# Autodesk Inventor assembly: Complete back top housing
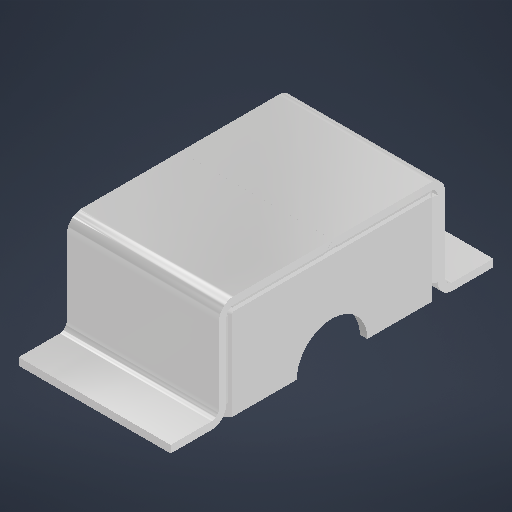
[picture p0: Inventor's stored thumbnail of the model, 512x512]
Saved by Autodesk Inventor 2026.3 (Build 303398000, 398)
## iProperties
Created: 2026-08-05
Part Number: Complete back top housing
Document SubType Name: Weldment
Designer: matot
Weld Material: Welded Aluminum-6061
Author: matot
## Documents named in this file (3)
- C:\Users\matot\OneDrive - Stellenbosch University\2026\MechatronicsProject478\Building the joint\Joint Assembly\Complete back top housing.iam
- C:\Users\matot\OneDrive - Stellenbosch University\2026\MechatronicsProject478\Building the joint\Joint Assembly\top front joint housing back.ipt
- C:\Users\matot\OneDrive - Stellenbosch University\2026\MechatronicsProject478\Building the joint\Joint Assembly\Bottom joint housing cover top back_ final.ipt
## Components (3 placed, 2 different names)
1. top front joint housing back:2 — Flush:1, Mate:1, Flush:2, Flush:3
2. top front joint housing back:3 — Flush:1, Mate:1, Flush:2, Flush:3, Mate:2, Mate:3, Flush:4
3. Bottom joint housing cover top back_ final:1 — Mate:2, Mate:3, Flush:4
## Relationships (7: Flush 4, Mate 3)
- Flush:1: top front joint housing back:2 ↔ top front joint housing back:3
- Mate:1: top front joint housing back:2 ↔ top front joint housing back:3
- Flush:2: top front joint housing back:2 ↔ top front joint housing back:3
- Flush:3: top front joint housing back:2 ↔ top front joint housing back:3
- Mate:2: top front joint housing back:3 ↔ Bottom joint housing cover top back_ final:1
- Mate:3: top front joint housing back:3 ↔ Bottom joint housing cover top back_ final:1
- Flush:4: top front joint housing back:3 ↔ Bottom joint housing cover top back_ final:1
